# Autodesk Inventor assembly: Assembly1_MIR
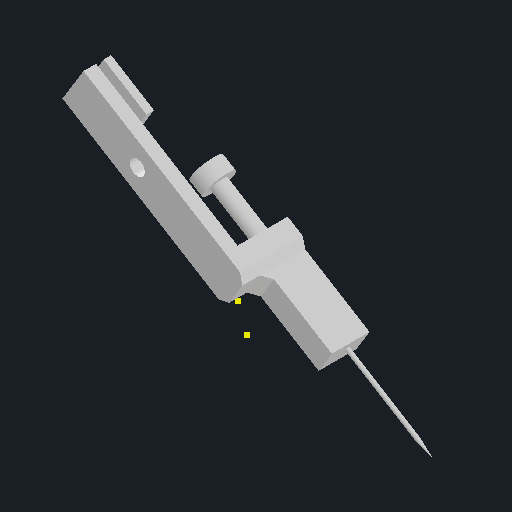
[picture p0: Inventor's stored thumbnail of the model, 512x512]
Saved by Autodesk Inventor 2026 (Build 300175050, 175E)
## iProperties
Created: 2025-06-30
Part Number: Assembly1_MIR
Document SubType Name: Assembly
Designer: Tobymegacat
Author: Tobymegacat
## Documents named in this file (4)
- C:\Users\herve\OneDrive\桌面\NIST\Inventor\Assembly1_MIR.iam
- C:\Users\herve\OneDrive\桌面\NIST\Inventor\Upper probe arm_MIR.ipt
- C:\Users\herve\OneDrive\桌面\NIST\Inventor\fake m3 screw_MIR.ipt
- C:\Users\herve\OneDrive\桌面\NIST\Inventor\fake needle_MIR.ipt
## Components (3 placed, 3 different names)
1. Upper probe arm_MIR:1 — Cylindrical:1
2. fake m3 screw_MIR:1 — Cylindrical:1, Rigid:1
3. fake needle_MIR:1 — Rigid:1
## Relationships (2: CylindricalJoint 1, WeldJoint 1)
- Cylindrical:1: Upper probe arm_MIR:1 ↔ fake m3 screw_MIR:1
- Rigid:1 [WeldJoint]: fake m3 screw_MIR:1 ↔ fake needle_MIR:1
